# Autodesk Inventor assembly: TR2 Arm
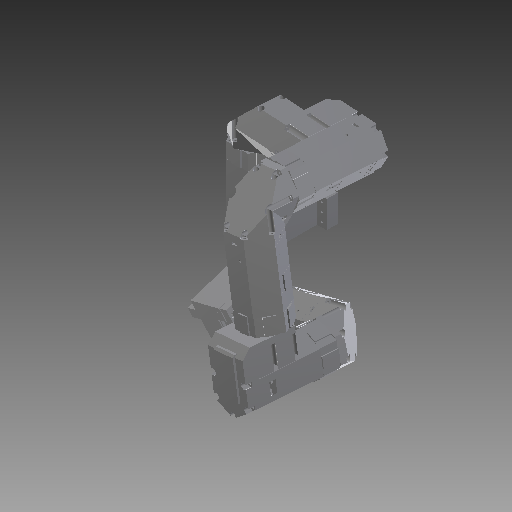
[picture p0: Inventor's stored thumbnail of the model, 512x512]
Saved by Autodesk Inventor 2017 SP1 (Build 210196100, 196)
## iProperties
Created: 2018-10-11
Part Number: TR2 Arm
Document SubType Name: Assembly
Designer: Zach
Author: Zach
## Documents named in this file (7)
- C:\Users\Zach\Documents\GitHub\tr2\Arm\Arm.iam
- C:\Users\Zach\Documents\GitHub\tr2\Arm\TARM09b.ipt
- C:\Users\Zach\Documents\GitHub\tr2\Arm\TARM01b.ipt
- C:\Users\Zach\Documents\GitHub\tr2\Arm\TARM02b.ipt
- C:\Users\Zach\Documents\GitHub\tr2\Arm\TARM14.ipt
- C:\Users\Zach\Documents\GitHub\tr2\Actuator 1.3\Actuator 1.3.iam
- C:\Users\Zach\Documents\GitHub\tr2\Gripper 1.1\Gripper 1.1.iam
## Components (12 placed, 6 different names)
1. TARM01b:1 — Mate:241, Mate:242, Mate:243, Mate:244, Mate:273, Mate:274
2. TARM09b:1 — Mate:186, Mate:187, Mate:188, Mate:249, Mate:250, Mate:251
3. TARM09b:2 — Mate:257, Mate:258, Mate:259, Mate:260, Mate:261
4. TARM02b:1 — Mate:186, Mate:187, Mate:188, Mate:247, Mate:248
5. TARM14:1 — Mate:252, Mate:253, Mate:254, Mate:255, Mate:256
6. TARM14:2 — Mate:262, Mate:263, Mate:264, Mate:265, Mate:266
7. Actuator 1.3:1 [sub-assembly] — Mate:244, Mate:247, Mate:248, Mate:273, Mate:274
8. Actuator 1.3:2 [sub-assembly] — Mate:249, Mate:250, Mate:251, Mate:252, Mate:253
9. Actuator 1.3:3 [sub-assembly] — Mate:254, Mate:255, Mate:256, Mate:257, Mate:258
10. Actuator 1.3:4 [sub-assembly] — Mate:259, Mate:260, Mate:261, Mate:262, Mate:263
11. Actuator 1.3:5 [sub-assembly] — Mate:264, Mate:265, Mate:266, Mate:270, Mate:272
12. Gripper 1.1:1 [sub-assembly] — Mate:270, Mate:272
## Relationships (31: Mate 31)
- Mate:186: TARM09b:1 ↔ TARM02b:1
- Mate:187: TARM09b:1 ↔ TARM02b:1
- Mate:188: TARM09b:1 ↔ TARM02b:1
- Mate:241: TARM01b:1
- Mate:242: TARM01b:1
- Mate:243: TARM01b:1
- Mate:244: TARM01b:1 ↔ Actuator 1.3:1
- Mate:247: TARM02b:1 ↔ Actuator 1.3:1
- Mate:248: TARM02b:1 ↔ Actuator 1.3:1
- Mate:249: TARM09b:1 ↔ Actuator 1.3:2
- Mate:250: TARM09b:1 ↔ Actuator 1.3:2
- Mate:251: TARM09b:1 ↔ Actuator 1.3:2
- Mate:252: TARM14:1 ↔ Actuator 1.3:2
- Mate:253: TARM14:1 ↔ Actuator 1.3:2
- Mate:254: TARM14:1 ↔ Actuator 1.3:3
- Mate:255: TARM14:1 ↔ Actuator 1.3:3
- Mate:256: TARM14:1 ↔ Actuator 1.3:3
- Mate:257: TARM09b:2 ↔ Actuator 1.3:3
- Mate:258: TARM09b:2 ↔ Actuator 1.3:3
- Mate:259: TARM09b:2 ↔ Actuator 1.3:4
- Mate:260: TARM09b:2 ↔ Actuator 1.3:4
- Mate:261: TARM09b:2 ↔ Actuator 1.3:4
- Mate:262: TARM14:2 ↔ Actuator 1.3:4
- Mate:263: TARM14:2 ↔ Actuator 1.3:4
- Mate:264: TARM14:2 ↔ Actuator 1.3:5
- Mate:265: TARM14:2 ↔ Actuator 1.3:5
- Mate:266: TARM14:2 ↔ Actuator 1.3:5
- Mate:270: Actuator 1.3:5 ↔ Gripper 1.1:1
- Mate:272: Actuator 1.3:5 ↔ Gripper 1.1:1
- Mate:273: TARM01b:1 ↔ Actuator 1.3:1
- Mate:274: TARM01b:1 ↔ Actuator 1.3:1
